# Autodesk Inventor assembly: gearbox
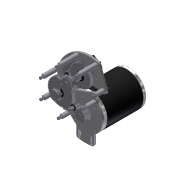
[picture p0: Inventor's stored thumbnail of the model, 180x180]
Saved by Autodesk Inventor 2012 (Build 160160000, 160)
## iProperties
Created: 2012-01-30
Part Number: gearbox
Document SubType Name: Assembly
Designer: Antonella Wilby
Author: Antonella Wilby
## Documents named in this file (42)
- C:\Users\Antonella\Documents\GCC Robotics 2012 - Mechanical\Robot 2.0\Drive Train\Gearbox\gearbox.iam
- C:\Users\Antonella\Documents\GCC Robotics 2012 - Mechanical\Robot 2.0\Drive Train\MY1020 Motor\my1020_motor.iam
- C:\Users\Antonella\Documents\GCC Robotics 2012 - Mechanical\Robot 2.0\Drive Train\Gearbox\standoff 2in.ipt
- C:\Users\Antonella\Documents\GCC Robotics 2012 - Mechanical\Robot 2.0\Drive Train\Gearbox\standoff 1.25in.ipt
- C:\Users\Antonella\Documents\GCC Robotics 2012 - Mechanical\Robot 2.0\Drive Train\Gearbox\fr8-zz.ipt
- C:\Users\Antonella\Documents\GCC Robotics 2012 - Mechanical\Robot 2.0\Drive Train\Gearbox\standoff 4.25in.ipt
- C:\Users\Antonella\Documents\GCC Robotics 2012 - Mechanical\Robot 2.0\Drive Train\Gearbox\fr6-zz.ipt
- C:\Users\Antonella\Documents\GCC Robotics 2012 - Mechanical\Robot 2.0\Drive Train\Gearbox\output_shaft.ipt
- C:\Users\Antonella\Documents\GCC Robotics 2012 - Mechanical\Robot 2.0\Drive Train\Gearbox\spur gear - 24t x 20dp x dd shaft.ipt
- C:\Users\Antonella\Documents\GCC Robotics 2012 - Mechanical\Robot 2.0\Drive Train\Gearbox\encoder mount.ipt
- C:\Users\Antonella\Documents\GCC Robotics 2012 - Mechanical\Robot 2.0\Electrical\encoder.ipt
- C:\Users\Antonella\Documents\GCC Robotics 2012 - Mechanical\Robot 2.0\Drive Train\Gearbox\spur gear -  60t x 20dp x 0.5 hexbore.ipt
- C:\Users\Antonella\Documents\GCC Robotics 2012 - Mechanical\Robot 2.0\Drive Train\Gearbox\spur gear - 14t x 20dp x 0.375 hexbore.ipt
- C:\Users\Antonella\Documents\GCC Robotics 2012 - Mechanical\Robot 2.0\Drive Train\Gearbox\output sprocket - No. 25 x 16t.ipt
- C:\Users\Antonella\Documents\GCC Robotics 2012 - Mechanical\Robot 2.0\Drive Train\Gearbox\spur gear - 50t x 20dp x 0.5 hexbore.ipt
- C:\Users\Antonella\Documents\GCC Robotics 2012 - Mechanical\Robot 2.0\Drive Train\Gearbox\spur gear - 50t x 20dp x 0.375 hexbore.ipt
- C:\Users\Antonella\Documents\GCC Robotics 2012 - Mechanical\Robot 2.0\Drive Train\Gearbox\shaft - step down No. 2 - 0.375 hex.ipt
- C:\Users\Antonella\Documents\GCC Robotics 2012 - Mechanical\Robot 2.0\Drive Train\Gearbox\shaft - step down No. 1 - 0.5 hex.ipt
- C:\Users\Antonella\Documents\GCC Robotics 2012 - Mechanical\Robot 2.0\Drive Train\Gearbox\spur gear - 19t x 20dp x 0.375 hexbore.ipt
- C:\Users\Antonella\Documents\GCC Robotics 2012 - Mechanical\Robot 2.0\Drive Train\Gearbox\back plate.ipt
- C:\Users\Antonella\Documents\GCC Robotics 2012 - Mechanical\Robot 2.0\Drive Train\Gearbox\motor plate.ipt
- C:\Users\Antonella\Documents\GCC Robotics 2012 - Mechanical\Robot 2.0\Drive Train\Gearbox\front plate.ipt
- C:\Users\Antonella\Documents\GCC Robotics 2012 - Mechanical\Robot 2.0\Drive Train\Gearbox\fr4.ipt
- C:\Users\Antonella\Documents\GCC Robotics 2012 - Mechanical\Robot 2.0\Drive Train\Gearbox\idler gear shaft.ipt
- C:\Users\Antonella\Documents\GCC Robotics 2012 - Mechanical\Robot 2.0\Drive Train\Gearbox\e-clip .375in shaft.ipt
- C:\Users\Antonella\Documents\GCC Robotics 2012 - Mechanical\Robot 2.0\Drive Train\Gearbox\e-clip .5in shaft.ipt
- C:\Users\Antonella\Documents\GCC Robotics 2012 - Mechanical\Robot 2.0\Drive Train\Gearbox\gearbox\Design Accelerator\Bolted Connection1.iam
- C:\Users\Antonella\Documents\GCC Robotics 2012 - Mechanical\Robot 2.0\Drive Train\Gearbox\gearbox\Design Accelerator\Bolted Connection2.iam
- C:\Users\Antonella\Documents\GCC Robotics 2012 - Mechanical\Robot 2.0\Drive Train\Gearbox\gearbox\Design Accelerator\Bolted Connection4.iam
- C:\Users\Antonella\Documents\GCC Robotics 2012 - Mechanical\Robot 2.0\Drive Train\Gearbox\gearbox\Design Accelerator\Bolted Connection5.iam
- C:\Users\Antonella\Documents\GCC Robotics 2012 - Mechanical\Robot 2.0\Drive Train\Gearbox\gearbox\Design Accelerator\Bolted Connection7.iam
- C:\Users\Antonella\Documents\GCC Robotics 2012 - Mechanical\Robot 2.0\Drive Train\Gearbox\gearbox\Design Accelerator\Bolted Connection8.iam
- C:\Users\Antonella\Documents\GCC Robotics 2012 - Mechanical\Robot 2.0\Drive Train\Gearbox\gearbox\Design Accelerator\Bolted Connection9.iam
- C:\Users\Antonella\Documents\GCC Robotics 2012 - Mechanical\Robot 2.0\Drive Train\Gearbox\gearbox\Design Accelerator\Bolted Connection10.iam
- C:\Users\Antonella\Documents\GCC Robotics 2012 - Mechanical\Robot 2.0\Drive Train\Gearbox\gearbox\Design Accelerator\Bolted Connection12.iam
- C:\Users\Antonella\Documents\GCC Robotics 2012 - Mechanical\Robot 2.0\Drive Train\Gearbox\gearbox\Design Accelerator\Bolted Connection13.iam
- C:\Users\Antonella\Documents\GCC Robotics 2012 - Mechanical\Robot 2.0\Drive Train\Gearbox\gearbox\Design Accelerator\Bolted Connection14.iam
- C:\Users\Antonella\Documents\GCC Robotics 2012 - Mechanical\Robot 2.0\Drive Train\Gearbox\gearbox\Design Accelerator\Bolted Connection15.iam
- C:\Users\Antonella\Documents\GCC Robotics 2012 - Mechanical\Robot 2.0\Drive Train\Gearbox\gearbox\Design Accelerator\Bolted Connection16.iam
- C:\Users\Antonella\Documents\GCC Robotics 2012 - Mechanical\Robot 2.0\Drive Train\Gearbox\gearbox\Design Accelerator\Bolted Connection17.iam
- C:\Users\Antonella\Documents\GCC Robotics 2012 - Mechanical\Robot 2.0\Drive Train\Gearbox\gearbox\Design Accelerator\Bolted Connection18.iam
- C:\Users\Antonella\Documents\GCC Robotics 2012 - Mechanical\Robot 2.0\Drive Train\Gearbox\gearbox\Design Accelerator\Bolted Connection19.iam
## Components (58 placed, 26 different names)
1. my1020_motor:1 [sub-assembly] — Mate:39, Mate:40, Flush:1, Mate:82, Mate:107, Mate:108, Mate:118
2. output_shaft:1 — Flush:3, Mate:58, Flush:76, Mate:77, Mate:99, Mate:100, Mate:164, Mate:165, Mate:166, Mate:167
3. encoder mount:1 — Mate:48, Mate:49, Flush:2, Mate:83, Mate:84, Mate:92
4. encoder:1 — Mate:48, Mate:49, Flush:2
5. Output Sprocket - 16 teeth — Flush:76, Mate:77, Mate:203
6. shaft - step down No. 2 - 0.375 hex:1 — Flush:63, Mate:64, Mate:65, Mate:66, Mate:103, Mate:104, Mate:160, Mate:161, Mate:168, Mate:169
7. shaft - step down No. 1 - 0.5 hex:1 — Mate:69, Mate:70, Flush:78, Mate:79, Mate:101, Mate:102, Mate:156, Mate:158, Mate:159, Mate:170
8. idler gear shaft:1 — Mate:145, Mate:146, Flush:147, Mate:148
9. back plate:1 — Mate:82, Mate:83, Mate:84, Mate:92, Mate:93, Mate:94, Mate:95, Mate:96, Mate:97, Mate:98, Mate:117, Mate:119, Mate:120, Mate:122, Mate:123, Mate:124, Mate:125, Mate:126, Mate:127, Mate:150, Mate:151, Mate:152, Mate:153, Mate:183, Mate:184, Mate:185, Mate:186, Mate:187, Mate:188, Mate:189, Mate:190
10. motor plate:1 — Mate:107, Mate:108, Mate:116, Mate:117, Mate:118, Mate:121, Mate:128, Mate:129, Mate:130, Mate:131, Mate:141, Mate:142, Mate:171, Mate:172, Mate:173, Mate:174, Mate:175, Mate:176, Mate:177, Mate:178, Mate:179, Mate:180, Mate:181, Mate:182
11. front plate:1 — Mate:132, Mate:134, Mate:135, Mate:136, Mate:137, Mate:138, Mate:139, Mate:140, Mate:143, Mate:144, Mate:191, Mate:192, Mate:193, Mate:194, Mate:195, Mate:196, Mate:197, Mate:198, Mate:199, Mate:200, Mate:201, Mate:202
12. Bolted Connection:5 [sub-assembly] — Mate:179, Mate:180
13. Bolted Connection:6 [sub-assembly] — Mate:181, Mate:182
14. standoff 4.25in:3 — Mate:150, Mate:151
15. standoff 4.25in:4 — Mate:152, Mate:153
16. standoff 2in:1 — Mate:122, Mate:123
17. standoff 2in:2 — Mate:119, Mate:120, Mate:121
18. standoff 1.25in:1 — Mate:130, Mate:131
19. standoff 1.25in:2 — Mate:128, Mate:129
20. standoff 4.25in:1 — Mate:126, Mate:127, Mate:132
21. standoff 4.25in:2 — Mate:124, Mate:125, Mate:134
22. fr4:1 — Mate:141, Mate:142, Mate:145, Mate:146, Mate:149
23. fr4:2 — Mate:143, Mate:144
24. fr8-zz:1 — Mate:93, Mate:94, Mate:99, Mate:100
25. fr8-zz:2 — Mate:135, Mate:136
26. fr8-zz:3 — Mate:139, Mate:140, Mate:203
27. fr6-zz:1 — Mate:95, Mate:96, Mate:101, Mate:102, Mate:106
28. fr6-zz:2 — Mate:97, Mate:98, Mate:103, Mate:104
29. fr6-zz:3 — Mate:137, Mate:138
30. Spur Gear 24t x dd shaft — Mate:39, Mate:40, Flush:1
31. Spur Gear 14t x .375 hex:2 — Flush:147, Mate:148, Mate:149
32. Spur Gear 60t x .5 hex — Mate:69, Mate:70, Mate:116
33. Spur Gear 19t x .375 hex — Flush:78, Mate:79, Flush:79, Mate:106
34. Spur Gear 50t x .375 hex — Mate:65, Mate:66, Mate:80, Flush:79
35. Spur Gear 14t x .375 hex — Flush:63, Mate:64, Mate:80, Flush:80
36. Spur Gear 50t x .5 hex — Flush:3, Mate:58, Flush:80
37. e-clip .5in shaft:1 — Mate:156, Mate:170
38. e-clip .5in shaft:2 — Mate:158, Mate:159
39. e-clip .375in shaft:2
40. e-clip .375in shaft:1
41. e-clip .375in shaft:3 — Mate:160, Mate:161
42. e-clip .375in shaft:4 — Mate:168, Mate:169
43. e-clip .5in shaft:3 — Mate:164, Mate:165
44. e-clip .5in shaft:4 — Mate:166, Mate:167
45. Bolted Connection:1 [sub-assembly] — Mate:171, Mate:172
46. Bolted Connection:2 [sub-assembly] — Mate:173, Mate:174
47. Bolted Connection:3 [sub-assembly] — Mate:175, Mate:176
48. Bolted Connection:4 [sub-assembly] — Mate:177, Mate:178
49. Bolted Connection:7 [sub-assembly] — Mate:183, Mate:184
50. Bolted Connection:8 [sub-assembly] — Mate:185, Mate:186
51. Bolted Connection:9 [sub-assembly] — Mate:187, Mate:188
52. Bolted Connection:10 [sub-assembly] — Mate:189, Mate:190
53. Bolted Connection:11 [sub-assembly] — Mate:191, Mate:192
54. Bolted Connection:12 [sub-assembly] — Mate:193, Mate:194
55. Bolted Connection:13 [sub-assembly] — Mate:195, Mate:196
56. Bolted Connection:14 [sub-assembly] — Mate:197, Mate:198
57. Bolted Connection:15 [sub-assembly] — Mate:199, Mate:200
58. Bolted Connection:16 [sub-assembly] — Mate:201, Mate:202
## Relationships (122: Mate 113, Flush 9)
- Mate:39: my1020_motor:1 ↔ Spur Gear 24t x dd shaft
- Mate:40: my1020_motor:1 ↔ Spur Gear 24t x dd shaft
- Flush:1 (1.5875 mm): my1020_motor:1 ↔ Spur Gear 24t x dd shaft
- Mate:48: encoder mount:1 ↔ encoder:1
- Mate:49: encoder mount:1 ↔ encoder:1
- Flush:2: encoder mount:1 ↔ encoder:1
- Flush:3: output_shaft:1 ↔ Spur Gear 50t x .5 hex
- Mate:58: output_shaft:1 ↔ Spur Gear 50t x .5 hex
- Flush:63: shaft - step down No. 2 - 0.375 hex:1 ↔ Spur Gear 14t x .375 hex
- Mate:64: shaft - step down No. 2 - 0.375 hex:1 ↔ Spur Gear 14t x .375 hex
- Mate:65: shaft - step down No. 2 - 0.375 hex:1 ↔ Spur Gear 50t x .375 hex
- Mate:66: shaft - step down No. 2 - 0.375 hex:1 ↔ Spur Gear 50t x .375 hex
- Mate:69: shaft - step down No. 1 - 0.5 hex:1 ↔ Spur Gear 60t x .5 hex
- Mate:70: shaft - step down No. 1 - 0.5 hex:1 ↔ Spur Gear 60t x .5 hex
- Flush:76: output_shaft:1 ↔ Output Sprocket - 16 teeth
- Mate:77: output_shaft:1 ↔ Output Sprocket - 16 teeth
- Flush:78: shaft - step down No. 1 - 0.5 hex:1 ↔ Spur Gear 19t x .375 hex
- Mate:79: shaft - step down No. 1 - 0.5 hex:1 ↔ Spur Gear 19t x .375 hex
- Mate:80: Spur Gear 50t x .375 hex ↔ Spur Gear 14t x .375 hex
- Flush:79 (-2.8765 mm): Spur Gear 19t x .375 hex ↔ Spur Gear 50t x .375 hex
- Flush:80 (-2.8575 mm): Spur Gear 14t x .375 hex ↔ Spur Gear 50t x .5 hex
- Mate:82: my1020_motor:1 ↔ back plate:1
- Mate:83: encoder mount:1 ↔ back plate:1
- Mate:84: encoder mount:1 ↔ back plate:1
- Mate:92: encoder mount:1 ↔ back plate:1
- Mate:93: back plate:1 ↔ fr8-zz:1
- Mate:94: back plate:1 ↔ fr8-zz:1
- Mate:95: back plate:1 ↔ fr6-zz:1
- Mate:96: back plate:1 ↔ fr6-zz:1
- Mate:97: back plate:1 ↔ fr6-zz:2
- Mate:98: back plate:1 ↔ fr6-zz:2
- Mate:99: output_shaft:1 ↔ fr8-zz:1
- Mate:100: output_shaft:1 ↔ fr8-zz:1
- Mate:101: shaft - step down No. 1 - 0.5 hex:1 ↔ fr6-zz:1
- Mate:102: shaft - step down No. 1 - 0.5 hex:1 ↔ fr6-zz:1
- Mate:103: shaft - step down No. 2 - 0.375 hex:1 ↔ fr6-zz:2
- Mate:104: shaft - step down No. 2 - 0.375 hex:1 ↔ fr6-zz:2
- Mate:106: fr6-zz:1 ↔ Spur Gear 19t x .375 hex
- Mate:107: my1020_motor:1 ↔ motor plate:1
- Mate:108: my1020_motor:1 ↔ motor plate:1
- Mate:116 (4.7625 mm): motor plate:1 ↔ Spur Gear 60t x .5 hex
- Mate:117: back plate:1 ↔ motor plate:1
- Mate:118: my1020_motor:1 ↔ motor plate:1
- Mate:119: back plate:1 ↔ standoff 2in:2
- Mate:120: back plate:1 ↔ standoff 2in:2
- Mate:121: motor plate:1 ↔ standoff 2in:2
- Mate:122: back plate:1 ↔ standoff 2in:1
- Mate:123: back plate:1 ↔ standoff 2in:1
- Mate:124: back plate:1 ↔ standoff 4.25in:2
- Mate:125: back plate:1 ↔ standoff 4.25in:2
- Mate:126: back plate:1 ↔ standoff 4.25in:1
- Mate:127: back plate:1 ↔ standoff 4.25in:1
- Mate:128: motor plate:1 ↔ standoff 1.25in:2
- Mate:129: motor plate:1 ↔ standoff 1.25in:2
- Mate:130: motor plate:1 ↔ standoff 1.25in:1
- Mate:131: motor plate:1 ↔ standoff 1.25in:1
- Mate:132: front plate:1 ↔ standoff 4.25in:1
- Mate:134: front plate:1 ↔ standoff 4.25in:2
- Mate:135: front plate:1 ↔ fr8-zz:2
- Mate:136: front plate:1 ↔ fr8-zz:2
- Mate:137: front plate:1 ↔ fr6-zz:3
- Mate:138: front plate:1 ↔ fr6-zz:3
- Mate:139: front plate:1 ↔ fr8-zz:3
- Mate:140: front plate:1 ↔ fr8-zz:3
- Mate:141: motor plate:1 ↔ fr4:1
- Mate:142: motor plate:1 ↔ fr4:1
- Mate:143: front plate:1 ↔ fr4:2
- Mate:144: front plate:1 ↔ fr4:2
- Mate:145: idler gear shaft:1 ↔ fr4:1
- Mate:146: idler gear shaft:1 ↔ fr4:1
- Flush:147: idler gear shaft:1 ↔ Spur Gear 14t x .375 hex:2
- Mate:148: idler gear shaft:1 ↔ Spur Gear 14t x .375 hex:2
- Mate:149: fr4:1 ↔ Spur Gear 14t x .375 hex:2
- Mate:150: back plate:1 ↔ standoff 4.25in:3
- Mate:151: back plate:1 ↔ standoff 4.25in:3
- Mate:152: back plate:1 ↔ standoff 4.25in:4
- Mate:153: back plate:1 ↔ standoff 4.25in:4
- Mate:156: shaft - step down No. 1 - 0.5 hex:1 ↔ e-clip .5in shaft:1
- Mate:158: shaft - step down No. 1 - 0.5 hex:1 ↔ e-clip .5in shaft:2
- Mate:159: shaft - step down No. 1 - 0.5 hex:1 ↔ e-clip .5in shaft:2
- Mate:160: shaft - step down No. 2 - 0.375 hex:1 ↔ e-clip .375in shaft:3
- Mate:161: shaft - step down No. 2 - 0.375 hex:1 ↔ e-clip .375in shaft:3
- Mate:164: output_shaft:1 ↔ e-clip .5in shaft:3
- Mate:165: output_shaft:1 ↔ e-clip .5in shaft:3
- Mate:166: output_shaft:1 ↔ e-clip .5in shaft:4
- Mate:167: output_shaft:1 ↔ e-clip .5in shaft:4
- Mate:168: shaft - step down No. 2 - 0.375 hex:1 ↔ e-clip .375in shaft:4
- Mate:169: shaft - step down No. 2 - 0.375 hex:1 ↔ e-clip .375in shaft:4
- Mate:170: shaft - step down No. 1 - 0.5 hex:1 ↔ e-clip .5in shaft:1
- Mate:171: motor plate:1 ↔ Bolted Connection:1
- Mate:172: motor plate:1 ↔ Bolted Connection:1
- Mate:173: motor plate:1 ↔ Bolted Connection:2
- Mate:174: motor plate:1 ↔ Bolted Connection:2
- Mate:175: motor plate:1 ↔ Bolted Connection:3
- Mate:176: motor plate:1 ↔ Bolted Connection:3
- Mate:177: motor plate:1 ↔ Bolted Connection:4
- Mate:178: motor plate:1 ↔ Bolted Connection:4
- Mate:179: motor plate:1 ↔ Bolted Connection:5
- Mate:180: motor plate:1 ↔ Bolted Connection:5
- Mate:181: motor plate:1 ↔ Bolted Connection:6
- Mate:182: motor plate:1 ↔ Bolted Connection:6
- Mate:183: back plate:1 ↔ Bolted Connection:7
- Mate:184: back plate:1 ↔ Bolted Connection:7
- Mate:185: back plate:1 ↔ Bolted Connection:8
- Mate:186: back plate:1 ↔ Bolted Connection:8
- Mate:187: back plate:1 ↔ Bolted Connection:9
- Mate:188: back plate:1 ↔ Bolted Connection:9
- Mate:189: back plate:1 ↔ Bolted Connection:10
- Mate:190: back plate:1 ↔ Bolted Connection:10
- Mate:191: front plate:1 ↔ Bolted Connection:11
- Mate:192: front plate:1 ↔ Bolted Connection:11
- Mate:193: front plate:1 ↔ Bolted Connection:12
- Mate:194: front plate:1 ↔ Bolted Connection:12
- Mate:195: front plate:1 ↔ Bolted Connection:13
- Mate:196: front plate:1 ↔ Bolted Connection:13
- Mate:197: front plate:1 ↔ Bolted Connection:14
- Mate:198: front plate:1 ↔ Bolted Connection:14
- Mate:199: front plate:1 ↔ Bolted Connection:15
- Mate:200: front plate:1 ↔ Bolted Connection:15
- Mate:201: front plate:1 ↔ Bolted Connection:16
- Mate:202: front plate:1 ↔ Bolted Connection:16
- Mate:203: Output Sprocket - 16 teeth ↔ fr8-zz:3
